# Autodesk Inventor assembly: scoomatic_halterung_bg
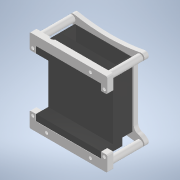
[picture p0: Inventor's stored thumbnail of the model, 180x180]
Saved by Autodesk Inventor 2021.3 (Build 253353010, 353A)
## iProperties
Created: 2021-07-26
Part Number: scoomatic_halterung_bg
Document SubType Name: Assembly
Designer: Markus
Author: Markus
## Documents named in this file (4)
- C:\Users\Markus\Documents\Inventor\Scoomatic-Jetson\scoomatic_halterung_bg.iam
- C:\Users\Markus\Documents\Inventor\Scoomatic-Jetson\jetson_dummy.ipt
- C:\Users\Markus\Documents\Inventor\Scoomatic-Jetson\Bauteil2.ipt
- C:\Users\Markus\Documents\Inventor\Scoomatic-Jetson\jetson_deckel.ipt
## Components (3 placed, 3 different names)
1. jetson_dummy:1 — Fluchtend:1, Fluchtend:2
2. Bauteil2:1 — Fluchtend:1
3. jetson_deckel:1 — Fluchtend:2
## Relationships (2: Flush 2)
- Fluchtend:1 [Flush]: jetson_dummy:1 ↔ Bauteil2:1
- Fluchtend:2 [Flush]: jetson_dummy:1 ↔ jetson_deckel:1
